# Autodesk Inventor assembly: HTPA30S3M060-A-N10_MIR_MIR_MIR1_MIR
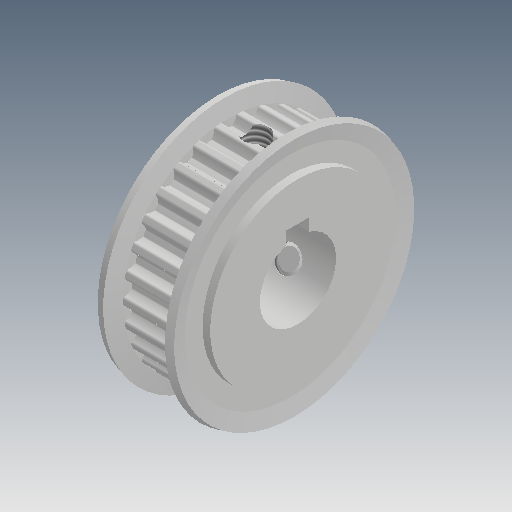
[picture p0: Inventor's stored thumbnail of the model, 512x512]
Saved by Autodesk Inventor 2020.5 (Build 245400000, 400)
## iProperties
Category: PARTsolutions
Company: MISUMI
Created: 2022-11-15
Part Number: HTPA30S3M060-A-N10_MIR_MIR_MIR1_MIR
Catalog Web Link: www.cadenas.de
Description: HTPA__S3M060, HTPA__S3M100, HTPA__S3M150, HTPB__S3M060, HTPB__S3M100, HTPB__S3M150, HTPK__S3M060, HTPK__S3M100, HTPK__S3M150, HTPN__S3M060, HTPN__S3M100, HTPN__S3M150, HTPT__S3M060, HTPT__S3M100, HTPT__S3M150, HTPM__S3M060, HTPM__S3M100, HTPM__S3M150, HTPP__S3M060, HTPP__S3M100, HTPP__S3M150, HTPS__S3M060, HTPS__S3M100, KHTPA__S3M060, KHTPA__S3M100, KHTPA__S3M150, KHTPK__S3M060, KHTPK__S3M100, KHTPK__S3M150-High Torque Timing Pulleys S3M Type
Vendor: MISUMI
Document SubType Name: Assembly
Designer: Administrator
Manufacturer: MISUMI
Mass: 5.3728 g
Surface Area: 37.292 cm^2
Volume: 5.3728 cm^3
Density: 1 g/cm^3
Title: HTPA30S3M060-A-N10
Author: Cadenas PARTsolutions
Comments: High Torque Timing Pulleys S3M Type
PSOL_IDENT_0: {$CADENAS_DATA/23d-libs/misumi/metric/51_timing_pulleys/htpk_s3m_asmtab.prj},844 {VTYP=3D},{STYP=ASS
PSOL_IDENT_1: TAB},{NB=HTPA30S3M060-A-N10},{LINA=HTPA30S3M060-A-N10},{NN=HTPA__S3M060, HTPA__S3M100, HTPA__S3M150,
PSOL_IDENT_2: HTPB__S3M060, HTPB__S3M100, HTPB__S3M150, HTPK__S3M060, HTPK__S3M100, HTPK__S3M150, HTPN__S3M060, H
PSOL_IDENT_3: TPN__S3M100, HTPN__S3M150, HTPT__S3M060, HTPT__S3M100, HTPT__S3M150, HTPM__S3M060, HTPM__S3M100, HTP
PSOL_IDENT_4: M__S3M150, HTPP__S3M060, HTPP__S3M100, HTPP__S3M150, HTPS__S3M060, HTPS__S3M100, KHTPA__S3M060, KHTP
PSOL_IDENT_5: A__S3M100, KHTPA__S3M150, KHTPK__S3M060, KHTPK__S3M100, KHTPK__S3M150},{DATE=28.10.2022 00:10:07},{G
PSOL_IDENT_6: EOMDATE=15.11.2021 05:07:15},{VERSION=},{LINEID=160},{WBVAR=MATP,ST,TNW,PS,SBS,DD,Z,J,Q,R,S,T,ALT1,A
PSOL_IDENT_7: LT2,M,QSC,QFC,QTC,ALT3,K,KSC,KFC,KTC,ALT4,ZM,ZSC,ZFC,ZTC,ALT5,ALT6,ALT7,FC,ALT8,SRG,ALT9,BTC,TL,ALT1
PSOL_IDENT_8: 0,TPC,ALT11,BC,ALT12,SLH,ALT13,BN},{WBNUMERIC=DD,Z,J,Q,R,S,T,QSC,QFC,QTC,K,KSC,KFC,KTC,ZSC,ZFC,ZTC,F
PSOL_IDENT_9: C,SRG,BTC,TL,BC,SLH,BN}  {NB=HTPA30S3M060-A-N10},{LINA=HTPA30S3M060-A-N10},{KT=DUMMY},{PN=HTPA30S3M0
PSOL_IDENT_10: 60-A-N10},{TYPE=HTPA},{MATP=A2017},{MATPALG='A2017','Aluminum Alloy 2000 series','S45C','1045 Carbon
PSOL_IDENT_11: Steel Equivalent','SUS304','304 Stainless Steel','A6000','6000 Series Aluminum Alloy'},{ST=CA},{STA
PSOL_IDENT_12: LG= 'CA','Clear Anodize','BA','Black Anodize','HAT','Hard Clear Anodize','ENP','Electroless Nickel P
PSOL_IDENT_13: lating' },{NT=30},{TNW=S3M060},{TNWALG= 'S3M060','S3M100','S3M150'    },{BW=6},{PS=A},{PSALG='A','B'
PSOL_IDENT_14: },{SBS=N},{SBSALG= 'H','Round Hole','P','Round Hole + Tap','N','New JIS Keywayed Bore + Tap (Standar
PSOL_IDENT_15: d)','NK','New JIS Keywayed Bore + Tap (width 4.0mm, height 1.8mm)','C','Old JIS Keywayed Bore + Tap'
PSOL_IDENT_16: ,'V','Stepped Hole', 'Y','Both Ends Stepped Hole','WB', 'Double Stepped Hole' },{SHSA= 'H','Round Ho
PSOL_IDENT_17: le','P','Round Hole + Tap','N','New JIS Keywayed Bore + Tap (Standard)','NK','New JIS Keywayed Bore
PSOL_IDENT_18: + Tap (width 4.0mm, height 1.8mm)','C','Old JIS Keywayed Bore + Tap','V','Stepped Hole', 'Y','Both E
PSOL_IDENT_19: nds Stepped Hole','WB', 'Double Stepped Hole' },{SHSB= 'H','Round Hole','P','Round Hole + Tap','N','
PSOL_IDENT_20: New JIS Keywayed Bore + Tap (Standard)','NK','New JIS Keywayed Bore + Tap (width 4.0mm, height 1.8mm
PSOL_IDENT_21: )','C','Old JIS Keywayed Bore + Tap','V','Stepped Hole', 'F','Stepped Hole (Counterbore holes on the
PSOL_IDENT_22: boss side)'},{SHSK= '','' },{SBSPN=-N10},{DD=10.00},{DDALG=[8:8/1],[10:14/1]},{DDHA=[6:6/1],6.35,[7
PSOL_IDENT_23: :12/1],12.7,[13:19/1]},{DDHBK=0},{DDPA=[6:6/1],6.35,[7:12/1],12.7,[13:19/1]},{DDPBK=0},{DDNA=[8:8/1]
PSOL_IDENT_24: ,[10:14/1]},{DDNBK=0},{DDNK=10},{DDCA=[10:10/1],[12:12/1]},{DDCBK=0},{DDVA=[6:6/1],6.35,[7:12/1],12.
PSOL_IDENT_25: 7,[13:17/1]},{DDVF=[6:6/1],6.35,[7:12/1],12.7,[13:14/1]},{DDY=[6:17/1]},{DDWB=[6:15/1]},{Z=0},{ZALG=
PSOL_IDENT_26: [0]},{ZQRMIN=12},{ZAMAX=19},{ZBMAX=16},{DDZ=10},{J=0.0},{JALG=[0]},{JMAX=9},{JMIN=2},{JPN=},{QRMAX=1
PSOL_IDENT_27: 9},{QRMIN=12},{WBRMAX=-2.00},{WBQMIN=14},{Q=0},{QALG=[0]},{QPN=},{R=0},{RALG=[0]},{S=0.0},{SALG=[0]}
PSOL_IDENT_28: ,{SPN=},{SMAX=5},{T=0.0},{TALG=[0]},{TPN=},{TMAX=8},{A=7},{W=11},{L=0},{PD=28.65},{OD=27.89},{D=0},{
PSOL_IDENT_29: DALG=20},{DE=23},{F=32},{E=23},{BBK=3.000},{TTK=1.4},{TT=1},{ANG=120},{WL=11},{ALT1=},{ALT1ALG= '','
PSOL_IDENT_30: w/o KC90 (Set Screw Angle)','KC90','with KC90 (Set Screw Angle)' },{ALT1PN=},{ALT2=},{ALT2ALG= '','N
PSOL_IDENT_31: ot applicable' },{M=N/A},{MALG= 'N/A' },{MFTALG= 'N/A' },{MSALG= 'N/A' },{M3D=0.000},{KDML=0},{ML=0}
PSOL_IDENT_32: ,{MUL=0},{PITCH=0},{QSC=0.0},{QSCALG=0},{QFC=0.0},{QFCALG=0},{QTC=0.0},{QTCALG=0},{QPCDMIN=0},{QPCDM
PSOL_IDENT_33: INALG=0},{QPCDMAX=19},{ALT2PN=},{ALT3=},{ALT3ALG= '','Not applicable' },{K=0.0},{KALG=0},{KMIN=4},{K
PSOL_IDENT_34: FTMAX=0.0},{KSMAX=0.0},{KSC=0.0},{KSCALG=0},{KFC=0.0},{KFCALG=0},{KTC=0.0},{KTCALG=0},{KPCDMIN=14},{
PSOL_IDENT_35: KPCDMINALG=14},{KPCDMAX=19},{KSCMIN=14.0},{KSCMINALG=14},{ALT3PN=},{ALT4=},{ALT4ALG= '','Not applica
PSOL_IDENT_36: ble' },{ALT4MIN=20.5},{ALT4MAX=12.5},{ZM=N/A},{ZMALG= 'N/A' },{ZMSALG= 'N/A' },{ZMFTALG= 'N/A' },{ZM
PSOL_IDENT_37: DD1=0.0},{ZMDD2=0.0},{ZMHH=0.0},{ZSC=0.0},{ZSCALG=[0]},{ZFC=0.0},{ZFCALG=[0]},{ZTC=0.0},{ZTCALG=[0]}
PSOL_IDENT_38: ,{ZPCDMIN=0},{ZPCDMINALG=0},{ZPCDMAX=19},{ALT4PN=},{ALT5=},{ALT5ALG= '','Flange Attached','NFC','wit
PSOL_IDENT_39: h NFC (Flange not Attached)' },{ALT5PN=},{ALT6=},{ALT6ALG= '','w/o Flange Attached on One Side Only'
PSOL_IDENT_40: ,'RFC','with RFC (Flange Attached on The Boss Side Only)','LFC','with LFC (Flange Attached on The Op
PSOL_IDENT_41: posite Side Only)' },{ALT6PN=},{ALT7=},{ALT7ALG= '','w/o FC (Flange Cut)','FC','with FC (Flange Cut)'
PSOL_IDENT_42: },{FC=0.0},{FCALG=0},{FCMIN=29.0},{FCMAX=30.0},{ALT7PN=},{ALT8=},{ALT8ALG= '','Not applicable' },{A
PSOL_IDENT_43: LT8ALGALG=19},{ALT8DD2=0},{ALT8MM=0},{ALT8NN=0},{QC=0},{KC=0},{ZC=0},{SRG=0.0},{SRGALG=[0]},{SRGMAX1=
PSOL_IDENT_44: 0},{SRGMAX=0},{DD2=0.0},{MM=0.00},{NN=0.00},{ALT8PN=},{ALT9ALG= '','Not applicable' },{ALT9=},{BTC9=
PSOL_IDENT_45: 11},{TL9=1},{BTC=0},{BTCALG=[0]},{TL=0.0},{TLALG=0},{TLMIN=1.0},{TLMAX=-11.5},{BTCL=0},{BTCD=0},{BTC
PSOL_IDENT_46: DALG=20.000},{ALT9PN=},{WLBCTL=11},{ALT10=},{ALT10ALG= '','w/o TPC (Tapped Hole Dimension)','TPC','w
PSOL_IDENT_47: ith TPC (Tapped Hole Dimension)' },{TPC=N/A},{TPCALG= 'N/A' },{TPCM=4},{ALT10PN=},{ALT11=},{ALT11ALG=
PSOL_IDENT_48: '','Not applicable' },{BC=0.0},{BCALG=0},{BCMIN=7},{BCMAX=-11.5},{BCPLANE=5.5},{M1WBC=5.5},{ALT11PN=
PSOL_IDENT_49: },{ALT12=},{ALT12ALG= '','w/o SLH (Set Screw Length)','SLH','with SLH (Set Screw Length)' },{SLH=0},
PSOL_IDENT_50: {SLHALG=[0]},{ALT12PN=},{AC=M4x3},{M1=4},{M1L=3},{TAP=0.000},{KYY=5},{KTT=8.945},{PLANE=11},{ALT13=}
PSOL_IDENT_51: ,{ALT13ALG= '', 'Not applicable' },{BN=0.0},{BNALG=0},{BNMIN=-10.5},{BNMAX=-1.0},{ALT13PN=},{PPATH=h
PSOL_IDENT_52: tpk_s3m/htpa_s3m_asmtpl.prj}
NB: HTPA30S3M060-A-N10
NN: 0
NT: 30
NBSYN: $PN.
LINA: HTPA30S3M060-A-N10
CATALOG: Misumi
PN: HTPA30S3M060-A-N10
MATP: Aluminum Alloy 2000 series
ST: Clear Anodize
TNW: S3M060
BW: 6
PS: A
SBS: New JIS Keywayed Bore + Tap (Standard)
DD: 10
Z: 0
J: 0
Q: 0
R: 0
S: 0
T: 0
A: 7
W: 11
L: 0
PD: 28.65
OD: 27.89
D: 0
F: 32
E: 23
TT: 1
ALT1: w/o KC90 (Set Screw Angle)
ALT2: Not applicable
M: N/A
QSC: 0
QFC: 0
QTC: 0
ALT3: Not applicable
K: 0
KSC: 0
KFC: 0
KTC: 0
ALT4: Not applicable
ZM: N/A
ZMDD1: 0
ZMDD2: 0
ZMHH: 0
ZSC: 0
ZFC: 0
ZTC: 0
ALT5: Flange Attached
ALT6: w/o Flange Attached on One Side Only
ALT7: w/o FC (Flange Cut)
FC: 0
ALT8: Not applicable
SRG: 0
DD2: 0
MM: 0
ALT9: Not applicable
BTC: 0
TL: 0
BTCL: 0
BTCD: 0
ALT10: w/o TPC (Tapped Hole Dimension)
TPC: N/A
ALT11: Not applicable
BC: 0
ALT12: w/o SLH (Set Screw Length)
SLH: 0
AC: M4x3
ALT13: Not applicable
BN: 0
SUPPLIER: MISUMI
ARTICLENO: HTPA30S3M060-A-N10
BOMINFO: HTPA30S3M060-A-N10
CREATOR: CADENAS GmbH
## Documents named in this file (3)
- C:\Users\Administrator\Documents\kamuy2\kamuy2\Parts\HTPA30S3M060-A-N10_Autodesk_Inventor_2020_20221115\AIS2020\HTPA30S3M060-A-N10_MIR_MIR_MIR1_MIR.iam
- C:\Users\Administrator\Documents\kamuy2\kamuy2\Parts\HTPA30S3M060-A-N10_Autodesk_Inventor_2020_20221115\AIS2020\HTPA30S3M060-A-N10_b_MIR_MIR_MIR1_MIR.ipt
- C:\Users\Administrator\Documents\kamuy2\kamuy2\Parts\HTPA30S3M060-A-N10_Autodesk_Inventor_2020_20221115\AIS2020\SET-SCREW4-3_MIR_MIR_MIR1_MIR.ipt
## Components (3 placed, 2 different names)
1. HTPA30S3M060-A-N10_b_MIR_MIR_MIR1_MIR:1 — to_screw1_XY@1 <-> CP_XY@2, to_screw1_Z@1 <-> CP_Z@2, to_screw2_XY@1 <-> CP_XY@3, to_screw2_Z@1 <-> CP_Z@3, to_screw1_YZ@1 <-> CP_YZ@2, to_screw2_YZ@1 <-> CP_YZ@3
2. SET-SCREW4-3_MIR_MIR_MIR1_MIR:1 — to_screw1_XY@1 <-> CP_XY@2, to_screw1_Z@1 <-> CP_Z@2, to_screw1_YZ@1 <-> CP_YZ@2
3. SET-SCREW4-3_MIR_MIR_MIR1_MIR:2 — to_screw2_XY@1 <-> CP_XY@3, to_screw2_Z@1 <-> CP_Z@3, to_screw2_YZ@1 <-> CP_YZ@3
## Relationships (6: Mate 4, Angle 2)
- to_screw1_XY@1 <-> CP_XY@2 [Mate]: HTPA30S3M060-A-N10_b_MIR_MIR_MIR1_MIR:1 ↔ SET-SCREW4-3_MIR_MIR_MIR1_MIR:1
- to_screw1_Z@1 <-> CP_Z@2 [Mate]: HTPA30S3M060-A-N10_b_MIR_MIR_MIR1_MIR:1 ↔ SET-SCREW4-3_MIR_MIR_MIR1_MIR:1
- to_screw2_XY@1 <-> CP_XY@3 [Mate]: HTPA30S3M060-A-N10_b_MIR_MIR_MIR1_MIR:1 ↔ SET-SCREW4-3_MIR_MIR_MIR1_MIR:2
- to_screw2_Z@1 <-> CP_Z@3 [Mate]: HTPA30S3M060-A-N10_b_MIR_MIR_MIR1_MIR:1 ↔ SET-SCREW4-3_MIR_MIR_MIR1_MIR:2
- to_screw1_YZ@1 <-> CP_YZ@2 [Angle] (0 deg): HTPA30S3M060-A-N10_b_MIR_MIR_MIR1_MIR:1 ↔ SET-SCREW4-3_MIR_MIR_MIR1_MIR:1
- to_screw2_YZ@1 <-> CP_YZ@3 [Angle] (0 deg): HTPA30S3M060-A-N10_b_MIR_MIR_MIR1_MIR:1 ↔ SET-SCREW4-3_MIR_MIR_MIR1_MIR:2
